# Autodesk Inventor assembly: 6in FIRST Wheel 2013 HiGrip
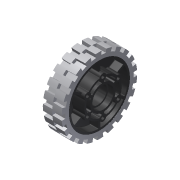
[picture p0: Inventor's stored thumbnail of the model, 180x180]
Saved by Autodesk Inventor 2013 (Build 170138000, 138)
## iProperties
Created: 2013-01-07
Part Number: 6in FIRST Wheel 2013 HiGrip
Document SubType Name: Assembly
Designer: Nemo
Author: Nemo
## Documents named in this file (3)
- H:\Nemo\Documents\Robotics\COTS Parts\Wheels\FIRST Wheels\6in FIRST Wheel 2013 HiGrip.iam
- H:\Nemo\Documents\Robotics\COTS Parts\Wheels\FIRST Wheels\Components\4in 2013 Hub.ipt
- H:\Nemo\Documents\Robotics\COTS Parts\Wheels\FIRST Wheels\Components\4 in tread.ipt
## Components (2 placed, 2 different names)
1. 4in 2013 Hub:1 — Mate:1, Mate:2
2. 4 in tread:1 — Mate:1, Mate:2
## Relationships (2: Mate 2)
- Mate:1: 4in 2013 Hub:1 ↔ 4 in tread:1
- Mate:2: 4in 2013 Hub:1 ↔ 4 in tread:1
